# Autodesk Inventor assembly: nozzle
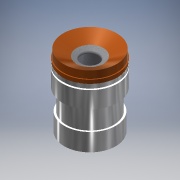
[picture p0: Inventor's stored thumbnail of the model, 180x180]
Saved by Autodesk Inventor 2017 SP1 (Build 210196100, 196)
## iProperties
Created: 2016-10-29
Part Number: nozzle
Document SubType Name: Assembly
Designer: cflannery
Author: cflannery
## Documents named in this file (7)
- D:\Triton_Rocket_Club\Propulsion\Launches\8-inch-flight\Design\CAD\Vehicle\Nozzle\trunk\nozzle.iam
- D:\Triton_Rocket_Club\Propulsion\Launches\8-inch-flight\Design\CAD\Vehicle\Nozzle\trunk\aluminum_casing.ipt
- D:\Triton_Rocket_Club\Propulsion\Launches\8-inch-flight\Design\CAD\Vehicle\Nozzle\trunk\aluminum_retainer.ipt
- D:\Triton_Rocket_Club\Propulsion\Launches\8-inch-flight\Design\CAD\Vehicle\Nozzle\trunk\aluminum_skirt.ipt
- D:\Triton_Rocket_Club\Propulsion\Launches\8-inch-flight\Design\CAD\Vehicle\Nozzle\trunk\graphite.ipt
- D:\Triton_Rocket_Club\Propulsion\Launches\8-inch-flight\Design\CAD\Vehicle\Nozzle\trunk\phenolic_bottom.ipt
- D:\Triton_Rocket_Club\Propulsion\Launches\8-inch-flight\Design\CAD\Vehicle\Nozzle\trunk\phenolic_top.ipt
## Components (6 placed, 6 different names)
1. aluminum_casing:1 — Mate:5, Mate:8, Mate:9, Mate:10
2. aluminum_retainer:1 — Mate:4, Mate:9
3. aluminum_skirt:1 — Mate:3, Mate:10
4. graphite:1 — Mate:1, Mate:2, Mate:3, Mate:4, Mate:5, Mate:6
5. phenolic_bottom:1 — Mate:1, Mate:7
6. phenolic_top:1 — Mate:2, Mate:6, Mate:7, Mate:8
## Relationships (10: Mate 10)
- Mate:1: graphite:1 ↔ phenolic_bottom:1
- Mate:2: graphite:1 ↔ phenolic_top:1
- Mate:3: aluminum_skirt:1 ↔ graphite:1
- Mate:4: aluminum_retainer:1 ↔ graphite:1
- Mate:5: aluminum_casing:1 ↔ graphite:1
- Mate:6: graphite:1 ↔ phenolic_top:1
- Mate:7: phenolic_bottom:1 ↔ phenolic_top:1
- Mate:8: aluminum_casing:1 ↔ phenolic_top:1
- Mate:9: aluminum_casing:1 ↔ aluminum_retainer:1
- Mate:10: aluminum_casing:1 ↔ aluminum_skirt:1
